# Autodesk Inventor assembly: Knifey Bit
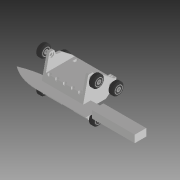
[picture p0: Inventor's stored thumbnail of the model, 180x180]
Saved by Autodesk Inventor 2020 (Build 240168000, 168)
## iProperties
Created: 2020-10-19
Part Number: Knifey Bit
Document SubType Name: Assembly
Designer: DDeGo
Author: DDeGo
## Documents named in this file (4)
- C:\Users\DDeGo\Documents\Drew\Projects\De-Cruster\cad\Knifey Bit.iam
- C:\Users\DDeGo\Documents\Drew\Projects\De-Cruster\cad\Knife Cart.ipt
- C:\Users\DDeGo\Documents\Drew\Projects\De-Cruster\cad\Knife.ipt
- C:\Users\DDeGo\Documents\Drew\Projects\De-Cruster\cad\VWheel.iam
## Components (8 placed, 3 different names)
1. Knife Cart:1 — Mate:2, Mate:4, Mate:5, Mate:6, Mate:7, Mate:8, Mate:9, Mate:10, Mate:11, Flush:5, Mate:12
2. Knife:1 — Mate:2, Flush:5, Mate:12
3. VWheel:1 [sub-assembly] — Flush:3, Mate:10
4. VWheel:2 [sub-assembly] — Flush:3, Flush:4, Mate:4, Mate:9
5. VWheel:3 [sub-assembly] — Flush:4, Mate:11
6. VWheel:4 [sub-assembly] — Flush:2, Mate:6
7. VWheel:5 [sub-assembly] — Flush:1, Mate:5, Mate:8
8. VWheel:6 [sub-assembly] — Flush:1, Flush:2, Mate:7
## Relationships (15: Mate 10, Flush 5)
- Mate:2: Knife Cart:1 ↔ Knife:1
- Flush:1: VWheel:5 ↔ VWheel:6
- Flush:2: VWheel:4 ↔ VWheel:6
- Flush:3: VWheel:1 ↔ VWheel:2
- Flush:4: VWheel:2 ↔ VWheel:3
- Mate:4 (6 mm): Knife Cart:1 ↔ VWheel:2
- Mate:5 (6 mm): Knife Cart:1 ↔ VWheel:5
- Mate:6: Knife Cart:1 ↔ VWheel:4
- Mate:7: Knife Cart:1 ↔ VWheel:6
- Mate:8: Knife Cart:1 ↔ VWheel:5
- Mate:9: Knife Cart:1 ↔ VWheel:2
- Mate:10: Knife Cart:1 ↔ VWheel:1
- Mate:11: Knife Cart:1 ↔ VWheel:3
- Flush:5 (25 mm): Knife Cart:1 ↔ Knife:1
- Mate:12: Knife Cart:1 ↔ Knife:1
